# Autodesk Inventor assembly: RS3-FullAs
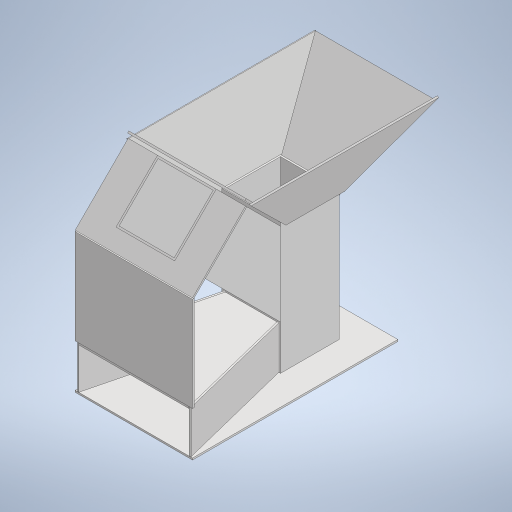
[picture p0: Inventor's stored thumbnail of the model, 512x512]
Saved by Autodesk Inventor 2024.3 (Build 283343000, 343)
## iProperties
Created: 2025-06-13
Part Number: RS3-FullAs
Document SubType Name: Assembly
Designer: ajclo
Author: ajclo
## Documents named in this file (10)
- C:\Users\ajclo\OneDrive - Stellenbosch University\Documents\BEng\Year IV\Skripsie\CAD\CAD Final Design\RS3-FullAs.iam
- C:\Users\ajclo\OneDrive - Stellenbosch University\Documents\BEng\Year IV\Skripsie\CAD\CAD Final Design\BottomPlateRS3.ipt
- C:\Users\ajclo\OneDrive - Stellenbosch University\Documents\BEng\Year IV\Skripsie\CAD\CAD Final Design\AI-TopPlateRS3.ipt
- C:\Users\ajclo\OneDrive - Stellenbosch University\Documents\BEng\Year IV\Skripsie\CAD\CAD Final Design\AI-SidePlateRS3.ipt
- C:\Users\ajclo\OneDrive - Stellenbosch University\Documents\BEng\Year IV\Skripsie\CAD\CAD Final Design\FLU-BackPlateRS3.ipt
- C:\Users\ajclo\OneDrive - Stellenbosch University\Documents\BEng\Year IV\Skripsie\CAD\CAD Final Design\FLU-SidePlatesRS3.ipt
- C:\Users\ajclo\OneDrive - Stellenbosch University\Documents\BEng\Year IV\Skripsie\CAD\CAD Final Design\FLU-ShaftRS3.ipt
- C:\Users\ajclo\OneDrive - Stellenbosch University\Documents\BEng\Year IV\Skripsie\CAD\CAD Final Design\WI-ShaftRS3.ipt
- C:\Users\ajclo\OneDrive - Stellenbosch University\Documents\BEng\Year IV\Skripsie\CAD\CAD Final Design\WI-CoverRS3.ipt
- C:\Users\ajclo\OneDrive - Stellenbosch University\Documents\BEng\Year IV\Skripsie\CAD\CAD Final Design\Front cover.ipt
## Components (12 placed, 9 different names)
1. BottomPlateRS3:1 — Mate:7, Mate:9, Mate:12, Flush:1, Mate:13, Flush:6
2. AI-TopPlateRS3:1 — Mate:6, Mate:8, Mate:10, Mate:11, Flush:3, Mate:16, Mate:20, Flush:5
3. AI-SidePlateRS3:1 — Mate:6, Mate:7, Mate:11, Mate:17
4. AI-SidePlateRS3:2 — Mate:8, Mate:9, Mate:10, Flush:3
5. FLU-BackPlateRS3:1
6. FLU-SidePlatesRS3:1
7. FLU-SidePlatesRS3:2
8. FLU-BackPlateRS3:2
9. FLU-ShaftRS3:1 — Mate:12, Flush:1, Mate:13, Mate:14, Flush:2, Mate:15, Mate:16, Mate:17
10. WI-ShaftRS3:1 — Mate:14, Flush:2, Mate:15, Flush:4, Mate:18, Mate:19
11. WI-CoverRS3:1 — Flush:4, Mate:18, Mate:19
12. Front cover:1 — Mate:20, Flush:5, Flush:6
## Relationships (21: Mate 15, Flush 6)
- Mate:6: AI-TopPlateRS3:1 ↔ AI-SidePlateRS3:1
- Mate:7: BottomPlateRS3:1 ↔ AI-SidePlateRS3:1
- Mate:8: AI-TopPlateRS3:1 ↔ AI-SidePlateRS3:2
- Mate:9: BottomPlateRS3:1 ↔ AI-SidePlateRS3:2
- Mate:10: AI-TopPlateRS3:1 ↔ AI-SidePlateRS3:2
- Mate:11: AI-TopPlateRS3:1 ↔ AI-SidePlateRS3:1
- Mate:12: BottomPlateRS3:1 ↔ FLU-ShaftRS3:1
- Flush:1: BottomPlateRS3:1 ↔ FLU-ShaftRS3:1
- Mate:13: BottomPlateRS3:1 ↔ FLU-ShaftRS3:1
- Mate:14: FLU-ShaftRS3:1 ↔ WI-ShaftRS3:1
- Flush:2: FLU-ShaftRS3:1 ↔ WI-ShaftRS3:1
- Mate:15: FLU-ShaftRS3:1 ↔ WI-ShaftRS3:1
- Flush:3: AI-TopPlateRS3:1 ↔ AI-SidePlateRS3:2
- Mate:16: AI-TopPlateRS3:1 ↔ FLU-ShaftRS3:1
- Mate:17: AI-SidePlateRS3:1 ↔ FLU-ShaftRS3:1
- Flush:4: WI-ShaftRS3:1 ↔ WI-CoverRS3:1
- Mate:18: WI-ShaftRS3:1 ↔ WI-CoverRS3:1
- Mate:19: WI-ShaftRS3:1 ↔ WI-CoverRS3:1
- Mate:20: AI-TopPlateRS3:1 ↔ Front cover:1
- Flush:5: AI-TopPlateRS3:1 ↔ Front cover:1
- Flush:6: BottomPlateRS3:1 ↔ Front cover:1
